# Autodesk Inventor assembly: eto
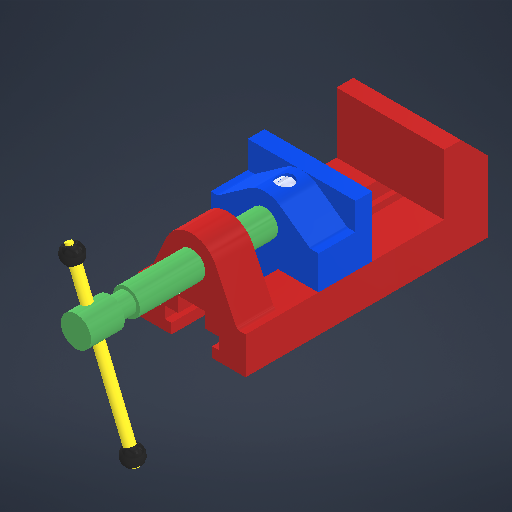
[picture p0: Inventor's stored thumbnail of the model, 512x512]
Saved by Autodesk Inventor 2025.4 (Build 294407000, 407)
## iProperties
Created: 2021-11-18
Part Number: eto
Description: STEP AP214
Document SubType Name: Assembly
Designer: VuQuan
Sending System: SolidWorks 2020
Preprocessor: SwSTEP 2.0
Title: eto.STEP
Revision Number: ANY
## Documents named in this file (10)
- D:\Edu\4CHaUI-Inventor\Assembly\b1\eto\eto.iam
- D:\Edu\4CHaUI-Inventor\Assembly\b1\eto\Bar Globes.ipt
- D:\Edu\4CHaUI-Inventor\Assembly\b1\eto\Base.ipt
- D:\Edu\4CHaUI-Inventor\Assembly\b1\eto\Base Plate.ipt
- D:\Edu\4CHaUI-Inventor\Assembly\b1\eto\Clamping Plate.ipt
- D:\Edu\4CHaUI-Inventor\Assembly\b1\eto\jaw screw.ipt
- D:\Edu\4CHaUI-Inventor\Assembly\b1\eto\Oval Fillister.ipt
- D:\Edu\4CHaUI-Inventor\Assembly\b1\eto\truc.ipt
- D:\Edu\4CHaUI-Inventor\Assembly\b1\eto\VICE.ipt
- D:\Edu\4CHaUI-Inventor\Assembly\b1\eto\ISO 2009 - M6 x 8 - 2.7 - ISO.ipt
## Components (16 placed, 11 different names)
1. Bar Globes_1 — Mate:9, Mate:10, Tangent:1
2. Base_2 — Mate:4, Flush:1, Mate:6, Mate:7, Mate:13, Insert:3, Insert:4, Insert:5, Insert:6
3. Base Plate_3 — Insert:3, Insert:4, Mate:22, Mate:23
4. Clamping Plate_4 — Insert:7, Insert:8
5. jaw screw_5 — Mate:3, Insert:1, Tangent:1
6. Oval Fillister_6 — Insert:2
7. truc_7 — Mate:3, Mate:9, Mate:10, Mate:11, Mate:12
8. VICE_8 — Mate:6, Mate:7, Mate:13, Insert:1, Insert:2, Insert:7, Insert:8, Mate:24, Mate:25
9. Bar Globes_9 — Mate:11, Mate:12
10. Base Plate_10 — Insert:5, Insert:6, Mate:21, Mate:26
11. ISO 2009 - M6 x 8 - 2.7 - ISO:2 — Mate:21
12. ISO 2009 - M6 x 8 - 2.7 - ISO:3 — Mate:22
13. ISO 2009 - M6 x 8 - 2.7 - ISO:4 — Mate:23
14. ISO 2009 - M6 x 8 - 2.7 - ISO:5 — Mate:24
15. ISO 2009 - M6 x 8 - 2.7 - ISO:6 — Mate:25
16. ISO 2009 - M6 x 8 - 2.7 - ISO:7 — Mate:26
## Relationships (25: Mate 15, Insert 8, Flush 1, Tangent 1)
- Mate:3: jaw screw_5 ↔ truc_7
- Mate:4: Base_2
- Flush:1: Base_2
- Mate:6: Base_2 ↔ VICE_8
- Mate:7: Base_2 ↔ VICE_8
- Mate:9: Bar Globes_1 ↔ truc_7
- Mate:10: Bar Globes_1 ↔ truc_7
- Mate:11: truc_7 ↔ Bar Globes_9
- Mate:12: truc_7 ↔ Bar Globes_9
- Mate:13: Base_2 ↔ VICE_8
- Insert:1: jaw screw_5 ↔ VICE_8
- Insert:2: Oval Fillister_6 ↔ VICE_8
- Insert:3: Base_2 ↔ Base Plate_3
- Insert:4: Base_2 ↔ Base Plate_3
- Insert:5: Base_2 ↔ Base Plate_10
- Insert:6: Base_2 ↔ Base Plate_10
- Insert:7: Clamping Plate_4 ↔ VICE_8
- Insert:8: Clamping Plate_4 ↔ VICE_8
- Tangent:1: Bar Globes_1 ↔ jaw screw_5
- Mate:21: Base Plate_10 ↔ ISO 2009 - M6 x 8 - 2.7 - ISO:2
- Mate:22: Base Plate_3 ↔ ISO 2009 - M6 x 8 - 2.7 - ISO:3
- Mate:23: Base Plate_3 ↔ ISO 2009 - M6 x 8 - 2.7 - ISO:4
- Mate:24: VICE_8 ↔ ISO 2009 - M6 x 8 - 2.7 - ISO:5
- Mate:25: VICE_8 ↔ ISO 2009 - M6 x 8 - 2.7 - ISO:6
- Mate:26: Base Plate_10 ↔ ISO 2009 - M6 x 8 - 2.7 - ISO:7
